# Autodesk Inventor assembly: assembledLinkage
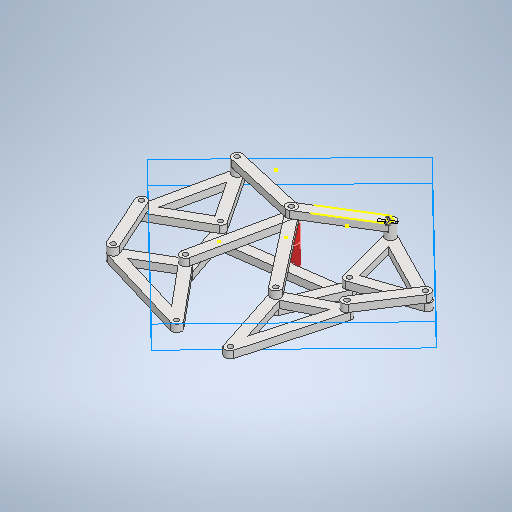
[picture p0: Inventor's stored thumbnail of the model, 512x512]
Saved by Autodesk Inventor 2026 (Build 300175050, 175E)
## iProperties
Created: 2025-05-24
Part Number: assembledLinkage
Document SubType Name: Assembly
Designer: omiye
Author: omiye
## Documents named in this file (10)
- C:\Projects\Arduino\strandbeest\assembledLinkage.iam
- C:\Projects\Arduino\strandbeest\f.ipt
- C:\Projects\Arduino\strandbeest\k.ipt
- C:\Projects\Arduino\strandbeest\c.ipt
- C:\Projects\Arduino\strandbeest\bde.ipt
- C:\Projects\Arduino\strandbeest\ghi.ipt
- C:\Projects\Arduino\strandbeest\j.ipt
- C:\Projects\Arduino\strandbeest\connector.ipt
- C:\Projects\Arduino\strandbeest\ghiMirror.ipt
- C:\Projects\Arduino\strandbeest\newM.ipt
## Components (14 placed, 9 different names)
1. f:1 — Mate:13, Mate:14, Mate:25, Mate:31
2. k:1 — Mate:5, Mate:16, Mate:23, Mate:30, Mate:58, Mate:61
3. c:1 — Mate:15, Mate:16, Mate:24, Mate:28, Mate:29
4. bde:1 — Mate:7, Mate:13, Mate:15, Flush:1, Mate:25, Mate:31
5. ghi:1 — Mate:5, Mate:14, Mate:23, Mate:24, Flush:1
6. j:1 — Mate:7, Mate:30, Mate:57, Mate:61
7. connector:1 — Mate:28, Mate:29, Mate:40, Mate:43, Mate:52, Mate:60
8. bde:2 — Mate:39, Mate:40, Mate:41, Mate:54, Mate:56
9. c:2 — Mate:43, Mate:52, Mate:53
10. f:2 — Mate:54, Mate:55, Mate:56
11. j:2 — Mate:36, Mate:37, Mate:39, Mate:41, Mate:57
12. k:2 — Mate:36, Mate:37, Mate:47, Mate:51, Mate:53, Mate:59
13. ghiMirror:1 — Mate:47, Mate:51, Mate:55
14. newM:1 — Mate:58, Mate:59, Mate:60
## Relationships (32: Mate 31, Flush 1)
- Mate:5: k:1 ↔ ghi:1
- Mate:7: bde:1 ↔ j:1
- Mate:13: f:1 ↔ bde:1
- Mate:14: f:1 ↔ ghi:1
- Mate:15: c:1 ↔ bde:1
- Mate:16: k:1 ↔ c:1
- Mate:23: k:1 ↔ ghi:1
- Mate:24: c:1 ↔ ghi:1
- Flush:1: bde:1 ↔ ghi:1
- Mate:25: f:1 ↔ bde:1
- Mate:28: c:1 ↔ connector:1
- Mate:29: c:1 ↔ connector:1
- Mate:30: k:1 ↔ j:1
- Mate:31: f:1 ↔ bde:1
- Mate:36: j:2 ↔ k:2
- Mate:37: j:2 ↔ k:2
- Mate:39: bde:2 ↔ j:2
- Mate:40: connector:1 ↔ bde:2
- Mate:41: bde:2 ↔ j:2
- Mate:43: connector:1 ↔ c:2
- Mate:47: k:2 ↔ ghiMirror:1
- Mate:51: k:2 ↔ ghiMirror:1
- Mate:52: connector:1 ↔ c:2
- Mate:53: c:2 ↔ k:2
- Mate:54: bde:2 ↔ f:2
- Mate:55: f:2 ↔ ghiMirror:1
- Mate:56: bde:2 ↔ f:2
- Mate:57: j:1 ↔ j:2
- Mate:58: k:1 ↔ newM:1
- Mate:59: k:2 ↔ newM:1
- Mate:60: connector:1 ↔ newM:1
- Mate:61: k:1 ↔ j:1
